# Autodesk Inventor assembly: Assembly2
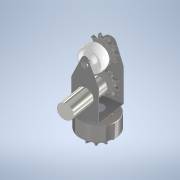
[picture p0: Inventor's stored thumbnail of the model, 180x180]
Saved by Autodesk Inventor 2020 (Build 240168000, 168)
## iProperties
Created: 2022-06-23
Part Number: Assembly2
Document SubType Name: Assembly
Designer: karimi2
Author: karimi2
## Documents named in this file (9)
- C:\Users\karimi2\Documents\PROJECT\Assembly2.iam
- C:\Users\karimi2\Documents\PROJECT\Frame.ipt
- C:\Users\karimi2\Documents\PROJECT\GearedDCmotor.ipt
- C:\Users\karimi2\Documents\PROJECT\casterwheel.ipt
- C:\Users\karimi2\Documents\PROJECT\wheelshaft.ipt
- C:\Users\karimi2\Documents\PROJECT\5mmSprocket.ipt
- C:\Users\karimi2\Documents\PROJECT\topshaft.ipt
- C:\Users\karimi2\Documents\PROJECT\Bearing.iam
- C:\Users\karimi2\Documents\PROJECT\19mmSprocket.ipt
## Components (9 placed, 8 different names)
1. Frame:1 — Mate:2, Mate:3, Flush:1, Mate:7, Mate:10, Mate:12, Mate:13, Mate:14, Flush:2
2. GearedDCmotor:1 — Mate:3, Flush:1, Mate:4, Mate:5
3. casterwheel:1 — Mate:2, Mate:6, Mate:9, Mate:10
4. 5mmSprocket:1 — Mate:4, Mate:5
5. wheelshaft:1 — Mate:6, Mate:7, Mate:9, Mate:11
6. 5mmSprocket:2 — Mate:11, Mate:12
7. topshaft:1 — Mate:13, Mate:14, Flush:2, Mate:15, Mate:16, Mate:17, Flush:3
8. Bearing:1 [sub-assembly] — Mate:15, Mate:16
9. 19mmSprocket:1 — Mate:17, Flush:3
## Relationships (18: Mate 15, Flush 3)
- Mate:2: Frame:1 ↔ casterwheel:1
- Mate:3: Frame:1 ↔ GearedDCmotor:1
- Flush:1 (-40 mm): Frame:1 ↔ GearedDCmotor:1
- Mate:4: GearedDCmotor:1 ↔ 5mmSprocket:1
- Mate:5 (-6 mm): GearedDCmotor:1 ↔ 5mmSprocket:1
- Mate:6: casterwheel:1 ↔ wheelshaft:1
- Mate:7: Frame:1 ↔ wheelshaft:1
- Mate:9: casterwheel:1 ↔ wheelshaft:1
- Mate:10 (8 mm): Frame:1 ↔ casterwheel:1
- Mate:11: wheelshaft:1 ↔ 5mmSprocket:2
- Mate:12 (9.519 mm): Frame:1 ↔ 5mmSprocket:2
- Mate:13: Frame:1 ↔ topshaft:1
- Mate:14: Frame:1 ↔ topshaft:1
- Flush:2: Frame:1 ↔ topshaft:1
- Mate:15: topshaft:1 ↔ Bearing:1
- Mate:16 (-35 mm): topshaft:1 ↔ Bearing:1
- Mate:17: topshaft:1 ↔ 19mmSprocket:1
- Flush:3: topshaft:1 ↔ 19mmSprocket:1
